# Autodesk Inventor assembly: 팔각형 OV-PAM 5패턴
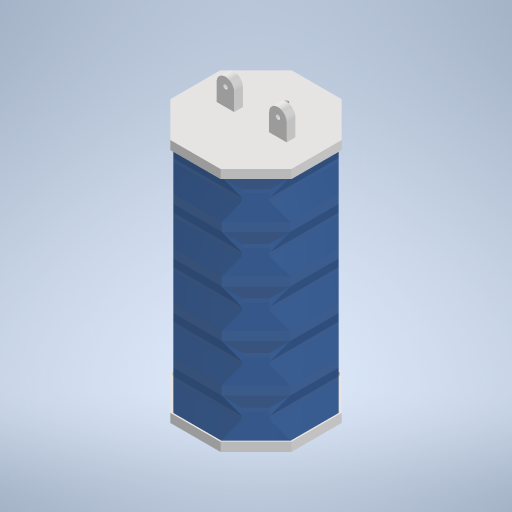
[picture p0: Inventor's stored thumbnail of the model, 512x512]
Saved by Autodesk Inventor 2024 (Build 280153000, 153)
## iProperties
Created: 2023-06-16
Part Number: 팔각형 OV-PAM 5패턴
Document SubType Name: Assembly
Designer: jsw
Author: jsw
## Documents named in this file (5)
- C:\승원\co-op\OV-PAM\팔각형 OV-PAM 5패턴.iam
- C:\승원\co-op\OV-PAM\팔각형 OV-PAM 5패턴 층 중단 하단 연결 층.ipt
- C:\승원\co-op\OV-PAM\팔각형 OV-PAM 5패턴 층 한개.ipt
- C:\승원\co-op\OV-PAM\팔각형 OV-PAM 5패턴 상단.ipt
- C:\승원\co-op\OV-PAM\팔각형 OV-PAM 5패턴 하단.ipt
## Components (7 placed, 4 different names)
1. 팔각형 OV-PAM 5패턴 층 중단 하단 연결 층:1 — 메이트:1, 플러쉬:1, 플러쉬:3, 메이트:3, 메이트:4, 메이트:5
2. 팔각형 OV-PAM 5패턴 층 중단 하단 연결 층:2 — 메이트:2, 플러쉬:5, 플러쉬:6, 메이트:6, 메이트:7, 메이트:8
3. 팔각형 OV-PAM 5패턴 상단:1 — 메이트:3, 메이트:4, 메이트:5
4. 팔각형 OV-PAM 5패턴 하단:1 — 메이트:6, 메이트:7, 메이트:8
5. 팔각형 OV-PAM 5패턴 층 한개:1 — 메이트:1, 플러쉬:1, 플러쉬:3
6. 팔각형 OV-PAM 5패턴 층 한개:2
7. 팔각형 OV-PAM 5패턴 층 한개:3 — 플러쉬:4, 메이트:2, 플러쉬:5, 플러쉬:6
## Component patterns: (3 elements, first: 팔각형 OV-PAM 5패턴 층 한개:1)
## Relationships (13: Mate 8, Flush 5)
- 메이트:1 [Mate]: 팔각형 OV-PAM 5패턴 층 중단 하단 연결 층:1 ↔ 팔각형 OV-PAM 5패턴 층 한개:1
- 플러쉬:1 [Flush]: 팔각형 OV-PAM 5패턴 층 중단 하단 연결 층:1 ↔ 팔각형 OV-PAM 5패턴 층 한개:1
- 플러쉬:3 [Flush]: 팔각형 OV-PAM 5패턴 층 중단 하단 연결 층:1 ↔ 팔각형 OV-PAM 5패턴 층 한개:1
- 플러쉬:4 [Flush] (-40.5 mm): 팔각형 OV-PAM 5패턴 층 한개:3
- 메이트:2 [Mate]: 팔각형 OV-PAM 5패턴 층 중단 하단 연결 층:2 ↔ 팔각형 OV-PAM 5패턴 층 한개:3
- 플러쉬:5 [Flush]: 팔각형 OV-PAM 5패턴 층 중단 하단 연결 층:2 ↔ 팔각형 OV-PAM 5패턴 층 한개:3
- 플러쉬:6 [Flush]: 팔각형 OV-PAM 5패턴 층 중단 하단 연결 층:2 ↔ 팔각형 OV-PAM 5패턴 층 한개:3
- 메이트:3 [Mate]: 팔각형 OV-PAM 5패턴 층 중단 하단 연결 층:1 ↔ 팔각형 OV-PAM 5패턴 상단:1
- 메이트:4 [Mate]: 팔각형 OV-PAM 5패턴 층 중단 하단 연결 층:1 ↔ 팔각형 OV-PAM 5패턴 상단:1
- 메이트:5 [Mate]: 팔각형 OV-PAM 5패턴 층 중단 하단 연결 층:1 ↔ 팔각형 OV-PAM 5패턴 상단:1
- 메이트:6 [Mate]: 팔각형 OV-PAM 5패턴 층 중단 하단 연결 층:2 ↔ 팔각형 OV-PAM 5패턴 하단:1
- 메이트:7 [Mate]: 팔각형 OV-PAM 5패턴 층 중단 하단 연결 층:2 ↔ 팔각형 OV-PAM 5패턴 하단:1
- 메이트:8 [Mate]: 팔각형 OV-PAM 5패턴 층 중단 하단 연결 층:2 ↔ 팔각형 OV-PAM 5패턴 하단:1
